# Autodesk Inventor assembly: RightMecanumDTAssemblyNewAttachment
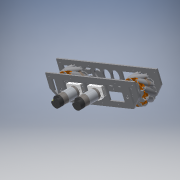
[picture p0: Inventor's stored thumbnail of the model, 180x180]
Saved by Autodesk Inventor 2017 (Build 210142000, 142)
## iProperties
Created: 2017-08-12
Part Number: RightMecanumDTAssemblyNewAttachment
Document SubType Name: Assembly
Designer: User
Author: User
## Documents named in this file (6)
- C:\Robotics\CAD\2016-17_CAD\DriveTrain\RightMecanumDTAssemblyNewAttachment.iam
- C:\Robotics\CAD\2016-17_CAD\DriveTrain\DriveTrainPlate2.0RightInside.ipt
- C:\Robotics\CAD\2016-17_CAD\DriveTrain\DriveTrainPlate2.0RightOutside.iam
- C:\Robotics\CAD\2016-17_CAD\DriveTrain\wheel sub assembly mechanum wheels .iam
- C:\Robotics\CAD\2016-17_CAD\DriveTrain\motor sub assembley.iam
- C:\Robotics\CAD\COTSParts\Tetrix\tetrix-motor-mounts-1.snapshot.1\Tetrex 2pc motor mount.ipt
## Components (8 placed, 5 different names)
1. DriveTrainPlate2.0RightInside:1 — Mate:6, Mate:7, Mate:8, Mate:9, Mate:10, Flush:3, Mate:11, Flush:4, Mate:13
2. DriveTrainPlate2.0RightOutside:1 [sub-assembly] — Flush:7, Mate:17, Mate:18
3. wheel sub assembly mechanum wheels :1 [sub-assembly] — Flush:3, Mate:11, Flush:6, Mate:17
4. wheel sub assembly mechanum wheels :2 [sub-assembly] — Flush:4, Mate:13, Flush:5, Flush:7, Mate:18
5. motor sub assembley:1 [sub-assembly] — Flush:6, Mate:16
6. motor sub assembley:2 [sub-assembly] — Flush:5, Mate:15
7. Tetrex 2pc motor mount:1 — Mate:9, Mate:10, Mate:16
8. Tetrex 2pc motor mount:2 — Mate:6, Mate:7, Mate:8, Mate:15
## Relationships (16: Mate 11, Flush 5)
- Mate:6: DriveTrainPlate2.0RightInside:1 ↔ Tetrex 2pc motor mount:2
- Mate:7: DriveTrainPlate2.0RightInside:1 ↔ Tetrex 2pc motor mount:2
- Mate:8: DriveTrainPlate2.0RightInside:1 ↔ Tetrex 2pc motor mount:2
- Mate:9: DriveTrainPlate2.0RightInside:1 ↔ Tetrex 2pc motor mount:1
- Mate:10: DriveTrainPlate2.0RightInside:1 ↔ Tetrex 2pc motor mount:1
- Flush:3: DriveTrainPlate2.0RightInside:1 ↔ wheel sub assembly mechanum wheels :1
- Mate:11: DriveTrainPlate2.0RightInside:1 ↔ wheel sub assembly mechanum wheels :1
- Flush:4: DriveTrainPlate2.0RightInside:1 ↔ wheel sub assembly mechanum wheels :2
- Mate:13: DriveTrainPlate2.0RightInside:1 ↔ wheel sub assembly mechanum wheels :2
- Flush:5: wheel sub assembly mechanum wheels :2 ↔ motor sub assembley:2
- Mate:15: motor sub assembley:2 ↔ Tetrex 2pc motor mount:2
- Flush:6: wheel sub assembly mechanum wheels :1 ↔ motor sub assembley:1
- Mate:16: motor sub assembley:1 ↔ Tetrex 2pc motor mount:1
- Flush:7: DriveTrainPlate2.0RightOutside:1 ↔ wheel sub assembly mechanum wheels :2
- Mate:17: DriveTrainPlate2.0RightOutside:1 ↔ wheel sub assembly mechanum wheels :1
- Mate:18: DriveTrainPlate2.0RightOutside:1 ↔ wheel sub assembly mechanum wheels :2
